# Autodesk Inventor assembly: Assembly_center_suspension
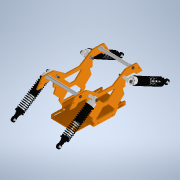
[picture p0: Inventor's stored thumbnail of the model, 180x180]
Saved by Autodesk Inventor 2020 (Build 240168000, 168)
## iProperties
Created: 2019-10-08
Part Number: Assembly_center_suspension
Document SubType Name: Assembly
Designer: maste
Author: maste
## Documents named in this file (8)
- C:\Users\maste\Documents\GitHub\autobot\robot_model\Assembly_center_suspension.iam
- C:\Users\maste\Documents\GitHub\autobot\robot_model\Assembly_center_unit.iam
- C:\Users\maste\Documents\GitHub\autobot\robot_model\RCT-H015_Tuerca_Conica.ipt
- C:\Users\maste\Documents\GitHub\autobot\robot_model\Ensamble_Amortiguador.iam
- C:\Users\maste\Documents\GitHub\autobot\robot_model\Assembly_center_suspension\Design Accelerator\cent_susp_BC001.iam
- C:\Users\maste\Documents\GitHub\autobot\robot_model\Assembly_center_suspension\Design Accelerator\cent_susp_BC002.iam
- C:\Users\maste\Documents\GitHub\autobot\robot_model\Assembly_center_suspension\Design Accelerator\cent_susp_BC003.iam
- C:\Users\maste\Documents\GitHub\autobot\robot_model\Assembly_center_suspension\Design Accelerator\cent_susp_BC004.iam
## Components (13 placed, 4 different names)
1. Assembly_center_unit:1 [sub-assembly] — Mate:1, Mate:2, Mate:3, Mate:4, Mate:5, Mate:6, Mate:7, Mate:8
2. RCT-H015_Tuerca_Conica:1 — Mate:1, Mate:2, Mate:9, Mate:10
3. RCT-H015_Tuerca_Conica:2 — Mate:3, Mate:4, Mate:13, Mate:14
4. RCT-H015_Tuerca_Conica:3 — Mate:5, Mate:6, Mate:15, Mate:16
5. RCT-H015_Tuerca_Conica:4 — Mate:7, Mate:8, Mate:11, Mate:12
6. Ensamble_Amortiguador:1 [sub-assembly] — Mate:9, Mate:10, Mate:19, Mate:20
7. Ensamble_Amortiguador:2 [sub-assembly] — Mate:13, Mate:14, Mate:17, Mate:18
8. Ensamble_Amortiguador:3 [sub-assembly] — Mate:15, Mate:16, Mate:21, Mate:22
9. Ensamble_Amortiguador:4 [sub-assembly] — Mate:11, Mate:12, Mate:23, Mate:24
10. Bolted Connection:1 [sub-assembly] — Mate:17, Mate:18
11. Bolted Connection:2 [sub-assembly] — Mate:19, Mate:20
12. Bolted Connection:3 [sub-assembly] — Mate:21, Mate:22
13. Bolted Connection:4 [sub-assembly] — Mate:23, Mate:24
## Relationships (24: Mate 24)
- Mate:1: Assembly_center_unit:1 ↔ RCT-H015_Tuerca_Conica:1
- Mate:2: Assembly_center_unit:1 ↔ RCT-H015_Tuerca_Conica:1
- Mate:3: Assembly_center_unit:1 ↔ RCT-H015_Tuerca_Conica:2
- Mate:4: Assembly_center_unit:1 ↔ RCT-H015_Tuerca_Conica:2
- Mate:5: Assembly_center_unit:1 ↔ RCT-H015_Tuerca_Conica:3
- Mate:6: Assembly_center_unit:1 ↔ RCT-H015_Tuerca_Conica:3
- Mate:7: Assembly_center_unit:1 ↔ RCT-H015_Tuerca_Conica:4
- Mate:8: Assembly_center_unit:1 ↔ RCT-H015_Tuerca_Conica:4
- Mate:9: RCT-H015_Tuerca_Conica:1 ↔ Ensamble_Amortiguador:1
- Mate:10: RCT-H015_Tuerca_Conica:1 ↔ Ensamble_Amortiguador:1
- Mate:11: RCT-H015_Tuerca_Conica:4 ↔ Ensamble_Amortiguador:4
- Mate:12: RCT-H015_Tuerca_Conica:4 ↔ Ensamble_Amortiguador:4
- Mate:13: RCT-H015_Tuerca_Conica:2 ↔ Ensamble_Amortiguador:2
- Mate:14: RCT-H015_Tuerca_Conica:2 ↔ Ensamble_Amortiguador:2
- Mate:15: RCT-H015_Tuerca_Conica:3 ↔ Ensamble_Amortiguador:3
- Mate:16: RCT-H015_Tuerca_Conica:3 ↔ Ensamble_Amortiguador:3
- Mate:17: Ensamble_Amortiguador:2 ↔ Bolted Connection:1
- Mate:18: Ensamble_Amortiguador:2 ↔ Bolted Connection:1
- Mate:19: Ensamble_Amortiguador:1 ↔ Bolted Connection:2
- Mate:20: Ensamble_Amortiguador:1 ↔ Bolted Connection:2
- Mate:21: Ensamble_Amortiguador:3 ↔ Bolted Connection:3
- Mate:22: Ensamble_Amortiguador:3 ↔ Bolted Connection:3
- Mate:23: Ensamble_Amortiguador:4 ↔ Bolted Connection:4
- Mate:24: Ensamble_Amortiguador:4 ↔ Bolted Connection:4
